# Autodesk Inventor assembly: ロボット
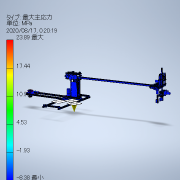
[picture p0: Inventor's stored thumbnail of the model, 180x180]
Saved by Autodesk Inventor 2020.3 (Build 243373000, 373)
## iProperties
Created: 2020-05-31
Part Number: ロボット
Document SubType Name: Assembly
Designer: totot
Mass: 3429.17 g
Surface Area: 13395.5 cm^2
Volume: 1595.28 cm^3
Density: 2.14957 g/cm^3
Author: totot
## Documents named in this file (12)
- D:\mysvn\ロボコン\キャチロボ\キャチロボ設計図\ロボット\ロボット.iam
- D:\mysvn\ロボコン\キャチロボ\キャチロボ設計図\ロボット\ロボットベース\ロボットベース.iam
- D:\mysvn\ロボコン\キャチロボ\キャチロボ設計図\ロボット\ロボット回転\ロボット回転.iam
- D:\mysvn\ロボコン\キャチロボ\キャチロボ設計図\ロボット\上下直動\上下直動.iam
- D:\mysvn\ロボコン\キャチロボ\キャチロボ設計図\ロボット\前後直動\前後直動.iam
- D:\mysvn\ロボコン\キャチロボ\キャチロボ設計図\ロボット\ハンド\ハンド.iam
- D:\mysvn\ロボコン\キャチロボ\キャチロボ設計図\ロボット\ロボット\AIP\FEA\dakpmi0qo.fins
- D:\mysvn\ロボコン\キャチロボ\キャチロボ設計図\ロボット\ロボット\AIP\FEA\dakpmi0qo.fsat
- D:\mysvn\ロボコン\キャチロボ\キャチロボ設計図\ロボット\ロボット\AIP\FEA\dakpmi0qo.ftes
- D:\mysvn\ロボコン\キャチロボ\キャチロボ設計図\ロボット\ロボット\AIP\FEA\dakpmi0qo.fwiz
- D:\mysvn\ロボコン\キャチロボ\キャチロボ設計図\ロボット\ロボット\AIP\FEA\dakpmi16o.fmsh
- D:\mysvn\ロボコン\キャチロボ\キャチロボ設計図\ロボット\ロボット\AIP\FEA\dakpmi16p.fres
## Components (5 placed, 5 different names)
1. 上下直動:1 [sub-assembly] — 挿入:1, 挿入:5, 挿入:6, 角度:1
2. 前後直動:1 [sub-assembly] — 挿入:1, 正接:1, 正接:2, 正接:3, 正接:4, フラッシュ:1
3. ロボットベース:1 [sub-assembly] — 挿入:2, 挿入:3, 挿入:4
4. ロボット回転:1 [sub-assembly] — 挿入:2, 挿入:3, 挿入:4, 正接:1, 正接:2, 正接:3, 正接:4, フラッシュ:1, 角度:1
5. ハンド:1 [sub-assembly] — 挿入:5, 挿入:6
## Relationships (12: Insert 6, Tangent 4, Flush 1, Angle 1)
- 挿入:1 [Insert] (-10 mm): 上下直動:1 ↔ 前後直動:1
- 挿入:2 [Insert]: ロボットベース:1 ↔ ロボット回転:1
- 挿入:3 [Insert]: ロボットベース:1 ↔ ロボット回転:1
- 挿入:4 [Insert]: ロボットベース:1 ↔ ロボット回転:1
- 正接:1 [Tangent]: 前後直動:1 ↔ ロボット回転:1
- 正接:2 [Tangent]: 前後直動:1 ↔ ロボット回転:1
- 正接:3 [Tangent]: 前後直動:1 ↔ ロボット回転:1
- 正接:4 [Tangent]: 前後直動:1 ↔ ロボット回転:1
- フラッシュ:1 [Flush]: 前後直動:1 ↔ ロボット回転:1
- 挿入:5 [Insert]: 上下直動:1 ↔ ハンド:1
- 挿入:6 [Insert]: 上下直動:1 ↔ ハンド:1
- 角度:1 [Angle] (0 deg): 上下直動:1 ↔ ロボット回転:1
